# Autodesk Inventor assembly: Ballscrew_Assembly
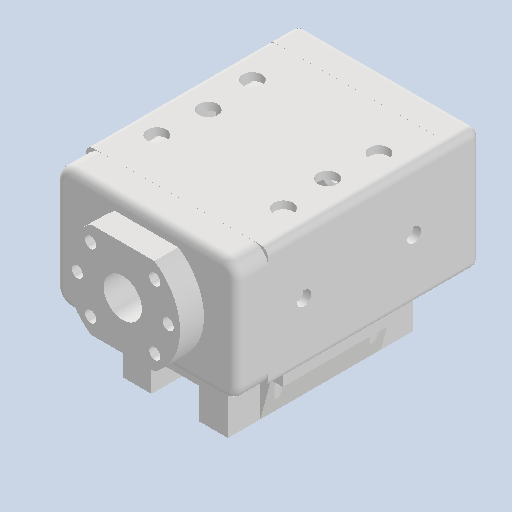
[picture p0: Inventor's stored thumbnail of the model, 512x512]
Saved by Autodesk Inventor 2023 (Build 270158000, 158)
## iProperties
Created: 2022-05-04
Part Number: Ballscrew_Assembly
Document SubType Name: Assembly
Designer: plebbb
Author: plebbb
## Documents named in this file (6)
- D:\Users\plebbb\Desktop\CNC_Project\Ballscrew_Assembly.iam
- D:\Users\plebbb\Desktop\CNC_Project\2x3_Tube_Short.ipt
- D:\Users\plebbb\Desktop\CNC_Project\2x3_Spacer.ipt
- D:\Users\plebbb\Desktop\CNC_Project\SFU1605_Nut.ipt
- D:\Users\plebbb\Desktop\CNC_Project\2x3_Spacer_Rear.ipt
- D:\Users\plebbb\Desktop\CNC_Project\HGW20CC_Slider.ipt
## Components (5 placed, 5 different names)
1. 2x3_Tube_Short:1
2. 2x3_Spacer:1
3. SFU1605_Nut:1
4. 2x3_Spacer_Rear:1
5. HGW20CC_Slider:1
## Relationships (12: Mate 8, Flush 4)
- [Mate]: 2x3_Spacer:1 ↔ SFU1605_Nut:1
- [Mate]: 2x3_Spacer:1 ↔ SFU1605_Nut:1
- [Mate]: 2x3_Spacer:1 ↔ SFU1605_Nut:1
- [Mate]: 2x3_Tube_Short:1 ↔ 2x3_Spacer:1
- [Flush]: 2x3_Tube_Short:1 ↔ 2x3_Spacer:1
- [Flush]: 2x3_Tube_Short:1 ↔ 2x3_Spacer:1
- [Mate]: 2x3_Tube_Short:1 ↔ 2x3_Spacer_Rear:1
- [Flush]: 2x3_Tube_Short:1 ↔ 2x3_Spacer_Rear:1
- [Flush]: 2x3_Tube_Short:1 ↔ 2x3_Spacer_Rear:1
- [Mate]: 2x3_Tube_Short:1 ↔ HGW20CC_Slider:1
- [Mate]: 2x3_Tube_Short:1 ↔ HGW20CC_Slider:1
- [Mate]: 2x3_Tube_Short:1 ↔ HGW20CC_Slider:1
## Named parameters: d0_d6 = 0 mm, d1_d7 = 0 mm, d2_d8 = 0 mm, d9_d11 = 0 mm
